# Autodesk Inventor assembly: Full_Design
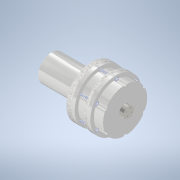
[picture p0: Inventor's stored thumbnail of the model, 180x180]
Saved by Autodesk Inventor 2022.3 (Build 263350000, 350)
## iProperties
Created: 2022-05-21
Part Number: Full_Design
Document SubType Name: Assembly
Designer: Mlees
Author: Mlees
## Documents named in this file (12)
- D:\504Engineering\Project_0000\Designs\Design_4\Full_Design.iam
- D:\504Engineering\Project_0000\Designs\Design_4\Created_Parts\Helion_Motor.ipt
- D:\504Engineering\Project_0000\Designs\Design_4\Created_Parts\Stage_1.ipt
- D:\504Engineering\Project_0000\Designs\Design_4\Created_Parts\Sun_Gear.ipt
- D:\504Engineering\Project_0000\Designs\Design_4\Downloaded_Parts\McMaster-Carr\91420A022_Steel Phillips Flat Head Screws.ipt
- D:\504Engineering\Project_0000\Designs\Design_4\Downloaded_Parts\McMaster-Carr\94180A321_Tapered Heat-Set Inserts for Plastic.ipt
- D:\504Engineering\Project_0000\Designs\Design_4\Created_Parts\Planet_Gear.ipt
- D:\504Engineering\Project_0000\Designs\Design_4\Created_Parts\Planet_Gear_Output.ipt
- D:\504Engineering\Project_0000\Designs\Design_4\Created_Parts\Stage_1_Lid.ipt
- D:\504Engineering\Project_0000\Designs\Design_4\Created_Parts\Stage_2.ipt
- D:\504Engineering\Project_0000\Designs\Design_4\Created_Parts\Stage_1_Output.ipt
- D:\504Engineering\Project_0000\Designs\Design_4\Downloaded_Parts\McMaster-Carr\91420A134_Steel Phillips Flat Head Screws.ipt
## Components (43 placed, 9 different names)
1. Helion_Motor:1 — Mate:1, Mate:2, Mate:3, Mate:4
2. Spur Gear2:1 — Mate:1, Mate:2, Mate:5, Mate:6, Mate:7, Mate:8, Mate:9, Mate:10, Mate:11, Mate:12, Mate:13, Mate:14, Mate:15, Mate:16, Mate:17, Mate:18, Mate:19, Mate:20, Mate:45, Mate:46, Mate:47, Mate:48, Mate:49, Mate:50, Mate:51, Mate:52
3. Spur Gear1:1 — Mate:3, Mate:4, Mate:64, Mate:65
4. 91420A022_Steel Phillips Flat Head Screws:1 — Mate:5, Mate:8
5. 91420A022_Steel Phillips Flat Head Screws:2 — Mate:6, Mate:7
6. 94180A321_Tapered Heat-Set Inserts for Plastic:1 — Mate:15, Mate:20
7. 94180A321_Tapered Heat-Set Inserts for Plastic:2 — Mate:11, Mate:12
8. 94180A321_Tapered Heat-Set Inserts for Plastic:3 — Mate:16, Mate:19
9. 94180A321_Tapered Heat-Set Inserts for Plastic:4 — Mate:17, Mate:18
10. 94180A321_Tapered Heat-Set Inserts for Plastic:5 — Mate:9, Mate:14
11. 94180A321_Tapered Heat-Set Inserts for Plastic:6 — Mate:10, Mate:13
12. Spur Gear2:2 — Mate:39, Mate:42, Mate:61, Mate:67
13. Spur Gear2:3 — Mate:38, Mate:43, Mate:62, Mate:66
14. Spur Gear2:4 — Mate:40, Mate:41, Mate:63, Mate:68
15. 94180A321_Tapered Heat-Set Inserts for Plastic:7 — Mate:55, Mate:59, Mate:61
16. 94180A321_Tapered Heat-Set Inserts for Plastic:8 — Mate:57, Mate:58, Mate:63
17. 94180A321_Tapered Heat-Set Inserts for Plastic:9 — Mate:56, Mate:60, Mate:62
18. 91420A022_Steel Phillips Flat Head Screws:3 — Mate:38, Mate:43
19. 91420A022_Steel Phillips Flat Head Screws:4 — Mate:39, Mate:42
20. 91420A022_Steel Phillips Flat Head Screws:5 — Mate:40, Mate:41
21. Stage_1_Lid:1 — Mate:45, Mate:46, Mate:53, Mate:54
22. 94180A321_Tapered Heat-Set Inserts for Plastic:10 — Mate:49, Mate:50
23. 94180A321_Tapered Heat-Set Inserts for Plastic:11 — Mate:51, Mate:52
24. 94180A321_Tapered Heat-Set Inserts for Plastic:12 — Mate:47, Mate:48
25. Spur Gear2:5 — Mate:53, Mate:54, Mate:90
26. Stage_1_Output:1 — Mate:55, Mate:56, Mate:57, Mate:58, Mate:59, Mate:60, Mate:64, Mate:65, Mate:66, Mate:67, Mate:68, Mate:87, Mate:88
27. Spur Gear2:6 — Mate:75, Mate:76, Mate:81, Mate:85
28. Spur Gear2:7 — Mate:77, Mate:78, Mate:82, Mate:86
29. Spur Gear2:8 — Mate:79, Mate:80, Mate:83, Mate:84
30. Planet_Gear_Output:1 — Mate:69, Mate:70, Mate:71, Mate:72, Mate:73, Mate:74, Mate:76, Mate:78, Mate:80, Mate:87, Mate:88, Mate:89
31. 91420A022_Steel Phillips Flat Head Screws:6 — Mate:81, Mate:85
32. 91420A022_Steel Phillips Flat Head Screws:7 — Mate:82, Mate:86
33. 91420A022_Steel Phillips Flat Head Screws:8 — Mate:83, Mate:84
34. 94180A321_Tapered Heat-Set Inserts for Plastic:13 — Mate:69, Mate:73, Mate:75
35. 94180A321_Tapered Heat-Set Inserts for Plastic:14 — Mate:70, Mate:72, Mate:79
36. 94180A321_Tapered Heat-Set Inserts for Plastic:15 — Mate:71, Mate:74, Mate:77
37. Stage_1_Lid:2 — Mate:89, Mate:90, Mate:91, Mate:92, Mate:93, Mate:94, Mate:95, Mate:96, Mate:97, Mate:98, Mate:99, Mate:100, Mate:101, Mate:102
38. 91420A134_Steel Phillips Flat Head Screws:1 — Mate:92, Mate:99
39. 91420A134_Steel Phillips Flat Head Screws:2 — Mate:91, Mate:98
40. 91420A134_Steel Phillips Flat Head Screws:3 — Mate:96, Mate:97
41. 91420A134_Steel Phillips Flat Head Screws:4 — Mate:93, Mate:100
42. 91420A134_Steel Phillips Flat Head Screws:5 — Mate:94, Mate:101
43. 91420A134_Steel Phillips Flat Head Screws:6 — Mate:95, Mate:102
## Relationships (84: Mate 84)
- Mate:1: Helion_Motor:1 ↔ Spur Gear2:1
- Mate:2: Helion_Motor:1 ↔ Spur Gear2:1
- Mate:3: Helion_Motor:1 ↔ Spur Gear1:1
- Mate:4: Helion_Motor:1 ↔ Spur Gear1:1
- Mate:5: Spur Gear2:1 ↔ 91420A022_Steel Phillips Flat Head Screws:1
- Mate:6: Spur Gear2:1 ↔ 91420A022_Steel Phillips Flat Head Screws:2
- Mate:7: Spur Gear2:1 ↔ 91420A022_Steel Phillips Flat Head Screws:2
- Mate:8: Spur Gear2:1 ↔ 91420A022_Steel Phillips Flat Head Screws:1
- Mate:9: Spur Gear2:1 ↔ 94180A321_Tapered Heat-Set Inserts for Plastic:5
- Mate:10: Spur Gear2:1 ↔ 94180A321_Tapered Heat-Set Inserts for Plastic:6
- Mate:11: Spur Gear2:1 ↔ 94180A321_Tapered Heat-Set Inserts for Plastic:2
- Mate:12: Spur Gear2:1 ↔ 94180A321_Tapered Heat-Set Inserts for Plastic:2
- Mate:13: Spur Gear2:1 ↔ 94180A321_Tapered Heat-Set Inserts for Plastic:6
- Mate:14: Spur Gear2:1 ↔ 94180A321_Tapered Heat-Set Inserts for Plastic:5
- Mate:15: Spur Gear2:1 ↔ 94180A321_Tapered Heat-Set Inserts for Plastic:1
- Mate:16: Spur Gear2:1 ↔ 94180A321_Tapered Heat-Set Inserts for Plastic:3
- Mate:17: Spur Gear2:1 ↔ 94180A321_Tapered Heat-Set Inserts for Plastic:4
- Mate:18: Spur Gear2:1 ↔ 94180A321_Tapered Heat-Set Inserts for Plastic:4
- Mate:19: Spur Gear2:1 ↔ 94180A321_Tapered Heat-Set Inserts for Plastic:3
- Mate:20: Spur Gear2:1 ↔ 94180A321_Tapered Heat-Set Inserts for Plastic:1
- Mate:38: Spur Gear2:3 ↔ 91420A022_Steel Phillips Flat Head Screws:3
- Mate:39: Spur Gear2:2 ↔ 91420A022_Steel Phillips Flat Head Screws:4
- Mate:40: Spur Gear2:4 ↔ 91420A022_Steel Phillips Flat Head Screws:5
- Mate:41: Spur Gear2:4 ↔ 91420A022_Steel Phillips Flat Head Screws:5
- Mate:42: Spur Gear2:2 ↔ 91420A022_Steel Phillips Flat Head Screws:4
- Mate:43: Spur Gear2:3 ↔ 91420A022_Steel Phillips Flat Head Screws:3
- Mate:45: Spur Gear2:1 ↔ Stage_1_Lid:1
- Mate:46: Spur Gear2:1 ↔ Stage_1_Lid:1
- Mate:47: Spur Gear2:1 ↔ 94180A321_Tapered Heat-Set Inserts for Plastic:12
- Mate:48: Spur Gear2:1 ↔ 94180A321_Tapered Heat-Set Inserts for Plastic:12
- Mate:49: Spur Gear2:1 ↔ 94180A321_Tapered Heat-Set Inserts for Plastic:10
- Mate:50: Spur Gear2:1 ↔ 94180A321_Tapered Heat-Set Inserts for Plastic:10
- Mate:51: Spur Gear2:1 ↔ 94180A321_Tapered Heat-Set Inserts for Plastic:11
- Mate:52: Spur Gear2:1 ↔ 94180A321_Tapered Heat-Set Inserts for Plastic:11
- Mate:53: Stage_1_Lid:1 ↔ Spur Gear2:5
- Mate:54: Stage_1_Lid:1 ↔ Spur Gear2:5
- Mate:55: 94180A321_Tapered Heat-Set Inserts for Plastic:7 ↔ Stage_1_Output:1
- Mate:56: 94180A321_Tapered Heat-Set Inserts for Plastic:9 ↔ Stage_1_Output:1
- Mate:57: 94180A321_Tapered Heat-Set Inserts for Plastic:8 ↔ Stage_1_Output:1
- Mate:58: 94180A321_Tapered Heat-Set Inserts for Plastic:8 ↔ Stage_1_Output:1
- Mate:59: 94180A321_Tapered Heat-Set Inserts for Plastic:7 ↔ Stage_1_Output:1
- Mate:60: 94180A321_Tapered Heat-Set Inserts for Plastic:9 ↔ Stage_1_Output:1
- Mate:61: Spur Gear2:2 ↔ 94180A321_Tapered Heat-Set Inserts for Plastic:7
- Mate:62: Spur Gear2:3 ↔ 94180A321_Tapered Heat-Set Inserts for Plastic:9
- Mate:63: Spur Gear2:4 ↔ 94180A321_Tapered Heat-Set Inserts for Plastic:8
- Mate:64: Spur Gear1:1 ↔ Stage_1_Output:1
- Mate:65: Spur Gear1:1 ↔ Stage_1_Output:1
- Mate:66: Spur Gear2:3 ↔ Stage_1_Output:1
- Mate:67: Spur Gear2:2 ↔ Stage_1_Output:1
- Mate:68: Spur Gear2:4 ↔ Stage_1_Output:1
- Mate:69: Planet_Gear_Output:1 ↔ 94180A321_Tapered Heat-Set Inserts for Plastic:13
- Mate:70: Planet_Gear_Output:1 ↔ 94180A321_Tapered Heat-Set Inserts for Plastic:14
- Mate:71: Planet_Gear_Output:1 ↔ 94180A321_Tapered Heat-Set Inserts for Plastic:15
- Mate:72: Planet_Gear_Output:1 ↔ 94180A321_Tapered Heat-Set Inserts for Plastic:14
- Mate:73: Planet_Gear_Output:1 ↔ 94180A321_Tapered Heat-Set Inserts for Plastic:13
- Mate:74: Planet_Gear_Output:1 ↔ 94180A321_Tapered Heat-Set Inserts for Plastic:15
- Mate:75: Spur Gear2:6 ↔ 94180A321_Tapered Heat-Set Inserts for Plastic:13
- Mate:76: Spur Gear2:6 ↔ Planet_Gear_Output:1
- Mate:77: Spur Gear2:7 ↔ 94180A321_Tapered Heat-Set Inserts for Plastic:15
- Mate:78: Spur Gear2:7 ↔ Planet_Gear_Output:1
- Mate:79: Spur Gear2:8 ↔ 94180A321_Tapered Heat-Set Inserts for Plastic:14
- Mate:80: Spur Gear2:8 ↔ Planet_Gear_Output:1
- Mate:81: Spur Gear2:6 ↔ 91420A022_Steel Phillips Flat Head Screws:6
- Mate:82: Spur Gear2:7 ↔ 91420A022_Steel Phillips Flat Head Screws:7
- Mate:83: Spur Gear2:8 ↔ 91420A022_Steel Phillips Flat Head Screws:8
- Mate:84: Spur Gear2:8 ↔ 91420A022_Steel Phillips Flat Head Screws:8
- Mate:85: Spur Gear2:6 ↔ 91420A022_Steel Phillips Flat Head Screws:6
- Mate:86: Spur Gear2:7 ↔ 91420A022_Steel Phillips Flat Head Screws:7
- Mate:87: Stage_1_Output:1 ↔ Planet_Gear_Output:1
- Mate:88: Stage_1_Output:1 ↔ Planet_Gear_Output:1
- Mate:89: Planet_Gear_Output:1 ↔ Stage_1_Lid:2
- Mate:90: Spur Gear2:5 ↔ Stage_1_Lid:2
- Mate:91: Stage_1_Lid:2 ↔ 91420A134_Steel Phillips Flat Head Screws:2
- Mate:92: Stage_1_Lid:2 ↔ 91420A134_Steel Phillips Flat Head Screws:1
- Mate:93: Stage_1_Lid:2 ↔ 91420A134_Steel Phillips Flat Head Screws:4
- Mate:94: Stage_1_Lid:2 ↔ 91420A134_Steel Phillips Flat Head Screws:5
- Mate:95: Stage_1_Lid:2 ↔ 91420A134_Steel Phillips Flat Head Screws:6
- Mate:96: Stage_1_Lid:2 ↔ 91420A134_Steel Phillips Flat Head Screws:3
- Mate:97: Stage_1_Lid:2 ↔ 91420A134_Steel Phillips Flat Head Screws:3
- Mate:98: Stage_1_Lid:2 ↔ 91420A134_Steel Phillips Flat Head Screws:2
- Mate:99: Stage_1_Lid:2 ↔ 91420A134_Steel Phillips Flat Head Screws:1
- Mate:100: Stage_1_Lid:2 ↔ 91420A134_Steel Phillips Flat Head Screws:4
- Mate:101: Stage_1_Lid:2 ↔ 91420A134_Steel Phillips Flat Head Screws:5
- Mate:102: Stage_1_Lid:2 ↔ 91420A134_Steel Phillips Flat Head Screws:6
